# Autodesk Inventor assembly: Slider-Crank_JacobMorgan_040915_pd3
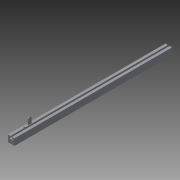
[picture p0: Inventor's stored thumbnail of the model, 180x180]
Saved by Autodesk Inventor 2015 (Build 190159000, 159)
## iProperties
Created: 2015-04-09
Part Number: Slider-Crank_JacobMorgan_040915_pd3
Document SubType Name: Assembly
Designer: WASHHSST
Author: WASHHSST
## Documents named in this file (3)
- C:\Users\washhsst\Documents\GitHub\myWork\Slider-Crank\Slider-Crank_JacobMorgan_040915_pd3.iam
- C:\Users\washhsst\Documents\GitHub\myWork\Slider-Crank\rail.ipt
- C:\Users\washhsst\Documents\GitHub\myWork\Slider-Crank\slider.ipt
## Components (2 placed, 2 different names)
1. rail:1 — Mate:1, Mate:2
2. slider:1 — Mate:1, Mate:2
## Relationships (2: Mate 2)
- Mate:1: rail:1 ↔ slider:1
- Mate:2: rail:1 ↔ slider:1
